# Autodesk Inventor assembly: Fairy Shell Spinner Assembly1
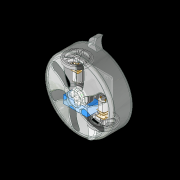
[picture p0: Inventor's stored thumbnail of the model, 180x180]
Saved by Autodesk Inventor 2022 (Build 260153000, 153)
## iProperties
Created: 2022-09-17
Part Number: Fairy Shell Spinner Assembly1
Document SubType Name: Assembly
Designer: tandu
Mass: 135.602 g
Surface Area: 677.555 cm^2
Volume: 80.2509 cm^3
Density: 1.68972 g/cm^3
Author: tandu
## Documents named in this file (7)
- C:\Users\tandu\Documents\GrabCAD\Fairyweights\Shell Spinner\Fairy Shell Spinner Assembly1.iam
- C:\Users\tandu\Documents\GrabCAD\Fairyweights\Shell Spinner\MicroGearmotor v3.ipt
- C:\Users\tandu\Documents\GrabCAD\Fairyweights\Shell Spinner\pololu-wheel-40x7mm-black.ipt
- C:\Users\tandu\Documents\GrabCAD\Fairyweights\Shell Spinner\DYS BE 1806 - Moteur complet.ipt
- C:\Users\tandu\Documents\GrabCAD\Fairyweights\Shell Spinner\2s 250mAh Mockup.ipt
- C:\Users\tandu\Documents\GrabCAD\Fairyweights\Shell Spinner\ShellSpinnerBottomPlate.ipt
- C:\Users\tandu\Documents\GrabCAD\Fairyweights\Shell Spinner\Shell.ipt
## Components (8 placed, 6 different names)
1. MicroGearmotor v3:1 — Insert:2, Flush:2, Mate:6, Mate:7
2. MicroGearmotor v3:2 — Insert:1, Flush:2, Flush:4, Mate:3, Mate:4, Mate:5
3. pololu-wheel-40x7mm-black:1 — Insert:1
4. pololu-wheel-40x7mm-black:2 — Insert:2
5. DYS BE 1806 - Moteur complet:1 — Insert:3, Insert:4, Insert:5
6. 2s 250mAh Mockup:1 — Flush:4
7. ShellSpinnerBottomPlate:1 — Mate:3, Mate:4, Mate:5, Mate:6, Mate:7, Insert:3, Insert:4
8. Shell:1 — Insert:5
## Relationships (12: Insert 5, Mate 5, Flush 2)
- Insert:1 (2.54 mm): MicroGearmotor v3:2 ↔ pololu-wheel-40x7mm-black:1
- Insert:2 (2.54 mm): MicroGearmotor v3:1 ↔ pololu-wheel-40x7mm-black:2
- Flush:2: MicroGearmotor v3:1 ↔ MicroGearmotor v3:2
- Flush:4: MicroGearmotor v3:2 ↔ 2s 250mAh Mockup:1
- Mate:3: MicroGearmotor v3:2 ↔ ShellSpinnerBottomPlate:1
- Mate:4: MicroGearmotor v3:2 ↔ ShellSpinnerBottomPlate:1
- Mate:5: MicroGearmotor v3:2 ↔ ShellSpinnerBottomPlate:1
- Mate:6: MicroGearmotor v3:1 ↔ ShellSpinnerBottomPlate:1
- Mate:7: MicroGearmotor v3:1 ↔ ShellSpinnerBottomPlate:1
- Insert:3: DYS BE 1806 - Moteur complet:1 ↔ ShellSpinnerBottomPlate:1
- Insert:4: DYS BE 1806 - Moteur complet:1 ↔ ShellSpinnerBottomPlate:1
- Insert:5: DYS BE 1806 - Moteur complet:1 ↔ Shell:1
